# Autodesk Inventor assembly: LeftMecanum-SubAssem01
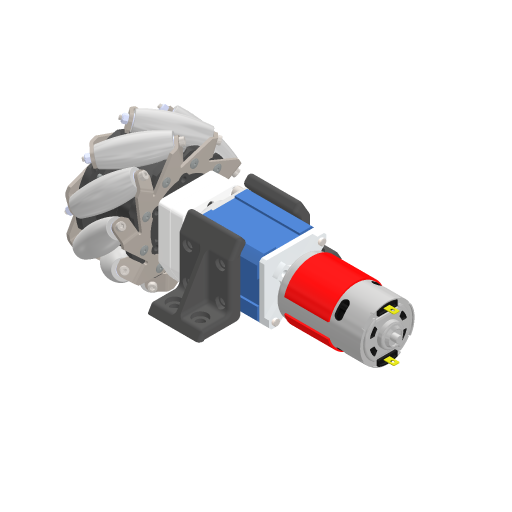
[picture p0: Inventor's stored thumbnail of the model, 512x512]
Saved by Autodesk Inventor 2024 (Build 280153000, 153)
## iProperties
Created: 2022-07-11
Part Number: LeftMecanum-SubAssem01
Document SubType Name: Assembly
Designer: Dave
Author: Dave
## Documents named in this file (8)
- C:\Autodesk\ChalkBot Github\ChalkbotMechanical\Chalkbot1.0\Chassis\V1\LeftMecanum-SubAssem01.iam
- C:\Autodesk\ChalkBot Github\ChalkbotMechanical\Chalkbot1.0\Chassis\V1\Mechanum STEP files\am-3775a AndyMark RedLine Motor (1).ipt
- C:\Autodesk\ChalkBot Github\ChalkbotMechanical\Chalkbot1.0\Chassis\V1\Motor and Gearbox STEP files\Hex Bore Mag Encoder Housing (217-6785).iam
- C:\Autodesk\ChalkBot Github\ChalkbotMechanical\Chalkbot1.0\Chassis\V1\Motor and Gearbox STEP files\am-3791 - 3000 x 500 Hex Shaft.ipt
- C:\Autodesk\ChalkBot Github\ChalkbotMechanical\Chalkbot1.0\Chassis\V1\Motor and Gearbox STEP files\2 Stage HD - 57 Sport.ipt
- C:\Autodesk\ChalkBot Github\ChalkbotMechanical\Chalkbot1.0\Chassis\V1\Mechanum STEP files\am-3918R 4HD 500H Mecanum Left.iam
- C:\Autodesk\ChalkBot Github\ChalkbotMechanical\Chalkbot1.0\Chassis\V1\Motor Mounts.ipt
- C:\Autodesk\ChalkBot Github\ChalkbotMechanical\Chalkbot1.0\Chassis\V1\Shaft Spacers.ipt
## Components (8 placed, 7 different names)
1. 2 Stage HD - 57 Sport:1 — Insert:4, Insert:5, Angle:1, Insert:6, Insert:7, Insert:8, Insert:9, Rotational:1, Cylindrical:1
2. am-3775a AndyMark RedLine Motor (1):1 — Insert:5
3. Hex Bore Mag Encoder Housing (217-6785):1 [sub-assembly] — Rotational:1, Rigid:1, Cylindrical:1
4. am-3791 - 3000 x 500 Hex Shaft:1 — Insert:4
5. am-3918R 4HD 500H Mecanum Left:1 [sub-assembly] — Rotational:2
6. Motor Mounts:1 — Insert:6, Insert:7
7. Motor Mounts:2 — Insert:8, Insert:9
8. Shaft Spacers:1 — Rigid:1, Rotational:2
## Relationships (14: Insert 9, RevoluteJoint 2, Angle 1, WeldJoint 1, CylindricalJoint 1)
- [Insert]: 2 Stage HD - 57 Sport:1 ↔ am-3775a AndyMark RedLine Motor (1):1
- [Insert]: 2 Stage HD - 57 Sport:1 ↔ am-3775a AndyMark RedLine Motor (1):1
- [Insert]: 2 Stage HD - 57 Sport:1 ↔ am-3791 - 3000 x 500 Hex Shaft:1
- Insert:4: 2 Stage HD - 57 Sport:1 ↔ am-3791 - 3000 x 500 Hex Shaft:1
- Insert:5: 2 Stage HD - 57 Sport:1 ↔ am-3775a AndyMark RedLine Motor (1):1
- Angle:1 (0 deg): 2 Stage HD - 57 Sport:1
- Insert:6: 2 Stage HD - 57 Sport:1 ↔ Motor Mounts:1
- Insert:7: 2 Stage HD - 57 Sport:1 ↔ Motor Mounts:1
- Insert:8: 2 Stage HD - 57 Sport:1 ↔ Motor Mounts:2
- Insert:9: 2 Stage HD - 57 Sport:1 ↔ Motor Mounts:2
- Rotational:1 [RevoluteJoint]: 2 Stage HD - 57 Sport:1 ↔ Hex Bore Mag Encoder Housing (217-6785):1
- Rigid:1 [WeldJoint]: Hex Bore Mag Encoder Housing (217-6785):1 ↔ Shaft Spacers:1
- Rotational:2 [RevoluteJoint]: am-3918R 4HD 500H Mecanum Left:1 ↔ Shaft Spacers:1
- Cylindrical:1: 2 Stage HD - 57 Sport:1 ↔ Hex Bore Mag Encoder Housing (217-6785):1
